# Autodesk Inventor assembly: Assembly2
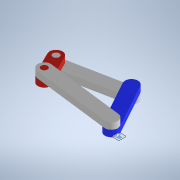
[picture p0: Inventor's stored thumbnail of the model, 180x180]
Saved by Autodesk Inventor 2022 (Build 260153000, 153)
## iProperties
Created: 2022-03-13
Part Number: Assembly2
Document SubType Name: Assembly
Designer: br4ch
Author: br4ch
## Documents named in this file (5)
- C:\Users\br4ch\M-and-Ms\Ansys labs\4 bar\Assembly2.iam
- C:\Users\br4ch\M-and-Ms\Ansys labs\4 bar\Part1.ipt
- C:\Users\br4ch\M-and-Ms\Ansys labs\4 bar\Part2.ipt
- C:\Users\br4ch\M-and-Ms\Ansys labs\4 bar\Part3.ipt
- C:\Users\br4ch\M-and-Ms\Ansys labs\4 bar\Part4.ipt
## Components (4 placed, 4 different names)
1. Part1:1 — Rotational:6, Rotational:9
2. Part2:1 — Rotational:8, Rotational:9
3. Part3:1 — Rotational:6, Rotational:7
4. Part4:1 — Rotational:7, Rotational:8
## Relationships (4: RevoluteJoint 4)
- Rotational:6 [RevoluteJoint]: Part1:1 ↔ Part3:1
- Rotational:7 [RevoluteJoint]: Part3:1 ↔ Part4:1
- Rotational:8 [RevoluteJoint]: Part2:1 ↔ Part4:1
- Rotational:9 [RevoluteJoint]: Part1:1 ↔ Part2:1
